# Autodesk Inventor assembly: TelescopeOptics
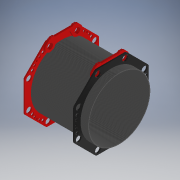
[picture p0: Inventor's stored thumbnail of the model, 180x180]
Saved by Autodesk Inventor 2022 (Build 260153000, 153)
## iProperties
Created: 2021-04-24
Part Number: TelescopeOptics
Document SubType Name: Assembly
Designer: Mick Veldhuis
Author: Mick Veldhuis
## Documents named in this file (3)
- C:\Users\Mick Veldhuis\Desktop\bsc-project\inventor\observatory\TelescopeOptics.iam
- C:\Users\Mick Veldhuis\Desktop\bsc-project\inventor\observatory\Primary.ipt
- C:\Users\Mick Veldhuis\Desktop\bsc-project\inventor\observatory\PlateConnector.ipt
## Components (3 placed, 2 different names)
1. Primary:1 — Tangent:1, Tangent:2
2. PlateConnector:1 — Tangent:1
3. PlateConnector:2 — Tangent:2
## Relationships (2: Tangent 2)
- Tangent:1: Primary:1 ↔ PlateConnector:1
- Tangent:2: Primary:1 ↔ PlateConnector:2
